# Autodesk Inventor assembly: 153
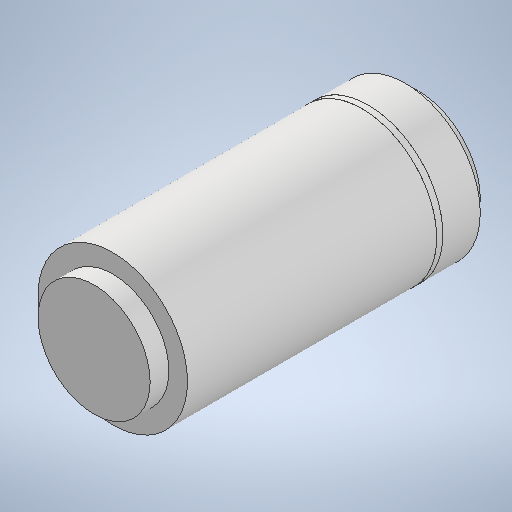
[picture p0: Inventor's stored thumbnail of the model, 512x512]
Saved by Autodesk Inventor 2025.1 (Build 291241000, 241)
## iProperties
Created: 2024-08-01
Part Number: 153
Document SubType Name: Assembly
Designer: ffogue
Author: ffogue
## Documents named in this file (4)
- C:\Projkete - Übungen\Freedom\153.iam
- C:\Projkete - Übungen\Freedom\153 part 1.ipt
- C:\Projkete - Übungen\Freedom\153 part 2.ipt
- C:\Projkete - Übungen\Freedom\sicherung153.ipt
## Components (3 placed, 3 different names)
1. 153 part 1:1 — Einfügen:1
2. 153 part 2:1 — Fluchtend:1
3. sicherung153:1 — Fluchtend:1, Einfügen:1
## Relationships (2: Flush 1, Insert 1)
- Fluchtend:1 [Flush]: 153 part 2:1 ↔ sicherung153:1
- Einfügen:1 [Insert]: 153 part 1:1 ↔ sicherung153:1
